# Autodesk Inventor assembly: 42146-00
(part 3 of 3)
- Einfügen:342 [Insert]: 67491-Yellow:12 ↔ 2780-Black:97
- Einfügen:343 [Insert]: 67491-Yellow:12 ↔ 2780-Black:99
- Einfügen:344 [Insert]: 67491-Yellow:12 ↔ 2780-Black:98
- Einfügen:345 [Insert]: 67491-Yellow:12 ↔ 6558-Blue:55
- Einfügen:346 [Insert]: 67491-Yellow:12 ↔ 6558-Blue:56
- Einfügen:347 [Insert]: 67491-Yellow:12 ↔ 6558-Blue:59
- Einfügen:348 [Insert]: 67491-Yellow:12 ↔ 6558-Blue:57
- Einfügen:349 [Insert]: 67491-Yellow:12 ↔ 6558-Blue:58
- Einfügen:350 [Insert]: 42146-20:1 ↔ 67491-Yellow:12
- Passend:154 [Mate]: 42146-20:1 ↔ 6558-Blue:55
- Einfügen:351 [Insert]: 2780-Black:100 ↔ 32525-Yellow:3
- Einfügen:352 [Insert]: 42146-20:1 ↔ 32525-Yellow:4
- Einfügen:353 [Insert]: 42146-20:1 ↔ 32525-Yellow:3
- Einfügen:354 [Insert]: 42146-25:1 ↔ 67491-Yellow:12
- Passend:155 [Mate]: 42146-25:1 ↔ 2780-Black:97
- Einfügen:355 [Insert]: 32054-LtBluishGray:23 ↔ 32524-Yellow:4
- Einfügen:356 [Insert]: 32054-LtBluishGray:24 ↔ 32524-Yellow:6
- Einfügen:357 [Insert]: 2780-Black:101 ↔ 771710-Black:3
- Einfügen:358 [Insert]: 2780-Black:102 ↔ 771710-Black:3
- Einfügen:359 [Insert]: 2780-Black:103 ↔ 771710-Black:3
- Einfügen:360 [Insert]: 6558-Blue:60 ↔ 18654-Black:2
- Einfügen:361 [Insert]: 2780-Black:104 ↔ 32524-Yellow:5
- Einfügen:362 [Insert]: 32524-Yellow:5 ↔ 18654-Black:2
- [Insert]: 6558-Blue:61 ↔ 18654-Black:3
- [Insert]: 2780-Black:105 ↔ 32524-Yellow:7
- [Insert]: 32524-Yellow:7 ↔ 18654-Black:3
- Einfügen:366 [Insert]: 42146-20:1 ↔ 32524-Yellow:4
- Einfügen:367 [Insert]: 42146-20:1 ↔ 32524-Yellow:6
- Passend:156 [Mate]: 42146-25:1 ↔ 32524-Yellow:6
- Passend:157 [Mate]: 42146-25:1 ↔ 32524-Yellow:4
- Einfügen:368 [Insert]: 67491-Yellow:12 ↔ 18654-Black:2
- Einfügen:369 [Insert]: 67491-Yellow:12 ↔ 18654-Black:3
- Einfügen:370 [Insert]: 42146-25:1 ↔ 771710-Black:3
- Passend:158 [Mate]: 42146-25:1 ↔ 2780-Black:101
- Passend:159 [Mate]: 2780-Black:104 ↔ 771710-Black:3
- Passend:160 [Mate]: 771710-Black:3 ↔ 2780-Black:105
- Einfügen:371 [Insert]: 42146-25:1 ↔ 67491-Yellow:13
- Passend:161 [Mate]: 42146-25:1 ↔ 67491-Yellow:13
- Einfügen:372 [Insert]: 771710-Black:1 ↔ 85824 - HUB:1
- Passend:162 [Mate]: 43093-Blue:15 ↔ 85824 - HUB:1
- Passend:163 [Mate]: 42146-24:1 ↔ 84428-LtBluishGray:1
- Passend:164 [Mate] (0.5 mm): 42146-24:1 ↔ 84428-LtBluishGray:1
- Passend:165 [Mate] (0.5 mm): 42146-24:1 ↔ 84428-LtBluishGray:1
- Passend:166 [Mate]: 84428-LtBluishGray:1 ↔ 84428-LtBluishGray:2
- Passend:167 [Mate]: 84428-LtBluishGray:1 ↔ 84428-LtBluishGray:2
- Passend:168 [Mate]: 84428-LtBluishGray:1 ↔ 84428-LtBluishGray:2
- [Mate]: 84428-LtBluishGray:3 ↔ 84428-LtBluishGray:4
- [Mate]: 84428-LtBluishGray:3 ↔ 84428-LtBluishGray:4
- [Mate]: 84428-LtBluishGray:3 ↔ 84428-LtBluishGray:4
- Passend:172 [Mate]: 84428-LtBluishGray:2 ↔ 84428-LtBluishGray:3
- Passend:173 [Mate]: 84428-LtBluishGray:2 ↔ 84428-LtBluishGray:3
- Passend:174 [Mate]: 84428-LtBluishGray:2 ↔ 84428-LtBluishGray:3
- [Mate]: 84428-LtBluishGray:5 ↔ 84428-LtBluishGray:6
- [Mate]: 84428-LtBluishGray:5 ↔ 84428-LtBluishGray:6
- [Mate]: 84428-LtBluishGray:5 ↔ 84428-LtBluishGray:6
- [Mate]: 84428-LtBluishGray:7 ↔ 84428-LtBluishGray:8
- [Mate]: 84428-LtBluishGray:7 ↔ 84428-LtBluishGray:8
- [Mate]: 84428-LtBluishGray:7 ↔ 84428-LtBluishGray:8
- [Mate]: 84428-LtBluishGray:6 ↔ 84428-LtBluishGray:7
- [Mate]: 84428-LtBluishGray:6 ↔ 84428-LtBluishGray:7
- [Mate]: 84428-LtBluishGray:6 ↔ 84428-LtBluishGray:7
- [Mate]: 84428-LtBluishGray:9 ↔ 84428-LtBluishGray:10
- [Mate]: 84428-LtBluishGray:9 ↔ 84428-LtBluishGray:10
- [Mate]: 84428-LtBluishGray:9 ↔ 84428-LtBluishGray:10
- [Mate]: 84428-LtBluishGray:11 ↔ 84428-LtBluishGray:12
- [Mate]: 84428-LtBluishGray:11 ↔ 84428-LtBluishGray:12
- [Mate]: 84428-LtBluishGray:11 ↔ 84428-LtBluishGray:12
- [Mate]: 84428-LtBluishGray:10 ↔ 84428-LtBluishGray:11
- [Mate]: 84428-LtBluishGray:10 ↔ 84428-LtBluishGray:11
- [Mate]: 84428-LtBluishGray:10 ↔ 84428-LtBluishGray:11
- Passend:193 [Mate]: 84428-LtBluishGray:5 ↔ 84428-LtBluishGray:12
- Passend:194 [Mate]: 84428-LtBluishGray:5 ↔ 84428-LtBluishGray:12
- Passend:195 [Mate]: 84428-LtBluishGray:5 ↔ 84428-LtBluishGray:12
- Passend:196 [Mate]: 84428-LtBluishGray:4 ↔ 84428-LtBluishGray:9
- Passend:197 [Mate]: 84428-LtBluishGray:4 ↔ 84428-LtBluishGray:9
- Passend:198 [Mate]: 84428-LtBluishGray:4 ↔ 84428-LtBluishGray:9
- [Mate]: 84428-LtBluishGray:13 ↔ 84428-LtBluishGray:14
- [Mate]: 84428-LtBluishGray:13 ↔ 84428-LtBluishGray:14
- [Mate]: 84428-LtBluishGray:13 ↔ 84428-LtBluishGray:14
- [Mate]: 84428-LtBluishGray:15 ↔ 84428-LtBluishGray:16
- [Mate]: 84428-LtBluishGray:15 ↔ 84428-LtBluishGray:16
- [Mate]: 84428-LtBluishGray:15 ↔ 84428-LtBluishGray:16
- [Mate]: 84428-LtBluishGray:14 ↔ 84428-LtBluishGray:15
- [Mate]: 84428-LtBluishGray:14 ↔ 84428-LtBluishGray:15
- [Mate]: 84428-LtBluishGray:14 ↔ 84428-LtBluishGray:15
- [Mate]: 84428-LtBluishGray:17 ↔ 84428-LtBluishGray:18
- [Mate]: 84428-LtBluishGray:17 ↔ 84428-LtBluishGray:18
- [Mate]: 84428-LtBluishGray:17 ↔ 84428-LtBluishGray:18
- [Mate]: 84428-LtBluishGray:19 ↔ 84428-LtBluishGray:20
- [Mate]: 84428-LtBluishGray:19 ↔ 84428-LtBluishGray:20
- [Mate]: 84428-LtBluishGray:19 ↔ 84428-LtBluishGray:20
- [Mate]: 84428-LtBluishGray:18 ↔ 84428-LtBluishGray:19
- [Mate]: 84428-LtBluishGray:18 ↔ 84428-LtBluishGray:19
- [Mate]: 84428-LtBluishGray:18 ↔ 84428-LtBluishGray:19
- [Mate]: 84428-LtBluishGray:21 ↔ 84428-LtBluishGray:22
- [Mate]: 84428-LtBluishGray:21 ↔ 84428-LtBluishGray:22
- [Mate]: 84428-LtBluishGray:21 ↔ 84428-LtBluishGray:22
- [Mate]: 84428-LtBluishGray:23 ↔ 84428-LtBluishGray:24
- [Mate]: 84428-LtBluishGray:23 ↔ 84428-LtBluishGray:24
- [Mate]: 84428-LtBluishGray:23 ↔ 84428-LtBluishGray:24
- [Mate]: 84428-LtBluishGray:22 ↔ 84428-LtBluishGray:23
- [Mate]: 84428-LtBluishGray:22 ↔ 84428-LtBluishGray:23
- [Mate]: 84428-LtBluishGray:22 ↔ 84428-LtBluishGray:23
- [Mate]: 84428-LtBluishGray:17 ↔ 84428-LtBluishGray:24
- [Mate]: 84428-LtBluishGray:17 ↔ 84428-LtBluishGray:24
- [Mate]: 84428-LtBluishGray:17 ↔ 84428-LtBluishGray:24
- [Mate]: 84428-LtBluishGray:16 ↔ 84428-LtBluishGray:21
- [Mate]: 84428-LtBluishGray:16 ↔ 84428-LtBluishGray:21
- [Mate]: 84428-LtBluishGray:16 ↔ 84428-LtBluishGray:21
- Passend:232 [Mate]: 42146-23:1 ↔ 84428-LtBluishGray:13
- Passend:233 [Mate] (0.5 mm): 42146-23:1 ↔ 84428-LtBluishGray:13
- Passend:234 [Mate] (0.5 mm): 42146-23:1 ↔ 84428-LtBluishGray:13
- Einfügen:373 [Insert]: 6558-Blue:63 ↔ 60484-Yellow:3
- Einfügen:374 [Insert]: 6558-Blue:62 ↔ 60484-Yellow:3
- Einfügen:375 [Insert]: 32073-LtBluishGray:3 ↔ 6536-Yellow:1
- Einfügen:376 [Insert]: 60484-Yellow:3 ↔ 6536-Yellow:1
- Einfügen:377 [Insert]: 60484-Yellow:3 ↔ 6536-Yellow:2
- Passend:235 [Mate]: 32073-LtBluishGray:3 ↔ 6536-Yellow:2
- Einfügen:378 [Insert]: 60484-Yellow:3 ↔ 79768-DkBluishGray:1
- Passend:236 [Mate]: 6558-Blue:63 ↔ 79768-DkBluishGray:1
- [Insert]: 60484-Yellow:4 ↔ 6536-Yellow:3
- Einfügen:380 [Insert]: 79768-DkBluishGray:1 ↔ 60484-Yellow:4
- Passend:237 [Mate]: 6558-Blue:62 ↔ 60484-Yellow:4
- Passend:238 [Mate]: 32073-LtBluishGray:3 ↔ 6536-Yellow:3
- Einfügen:381 [Insert]: 42146-22:1 ↔ 6536-Yellow:1
- Passend:239 [Mate]: 42146-22:1 ↔ 6536-Yellow:3
- Einfügen:382 [Insert]: 42146-22:1 ↔ 77765-MediumStoneGrey:8
- Einfügen:383 [Insert]: 42146-22:1 ↔ 77765-MediumStoneGrey:7
- Einfügen:384 [Insert]: 42146-22:1 ↔ 77765-MediumStoneGrey:9
- Einfügen:385 [Insert]: 42146-22:1 ↔ 32525-LtBluishGray:1
- Passend:240 [Mate]: 42146-22:1 ↔ 32525-LtBluishGray:1
- Einfügen:386 [Insert]: 42146-20:1 ↔ 32054-LtBluishGray:26
- Einfügen:387 [Insert]: 42146-20:1 ↔ 32054-LtBluishGray:25
- Einfügen:388 [Insert]: 42146-20:1 ↔ 42146-26:1
- Einfügen:389 [Insert]: 67498-shock absorber:2 ↔ 2780-Black:106
- Einfügen:390 [Insert]: 67498-shock absorber:2 ↔ 2780-Black:109
- Einfügen:391 [Insert]: 67498-shock absorber:1 ↔ 2780-Black:108
- Einfügen:392 [Insert]: 67498-shock absorber:1 ↔ 2780-Black:107
- Einfügen:393 [Insert]: 67498-shock absorber:2 ↔ 32525-Yellow:3
- Einfügen:394 [Insert]: 67498-shock absorber:1 ↔ 32525-Yellow:4
- Passend:241 [Mate]: 32525-Yellow:4 ↔ 2780-Black:108
- Passend:242 [Mate]: 32525-Yellow:3 ↔ 2780-Black:106
- Passend:243 [Mate]: 42146-26:1 ↔ 67498-shock absorber:2
- Passend:244 [Mate]: 42146-26:1 ↔ 67498-shock absorber:1
- Passend:245 [Mate]: 42146-26:1 ↔ 42146-27:1
- Einfügen:396 [Insert]: 42146-27:1 ↔ 44294-Yellow:1
- Einfügen:397 [Insert]: 42146-27:1 ↔ 44294-Yellow:2
- Einfügen:398 [Insert]: 6632-LtBluishGray:1 ↔ 32062-Red:1
- Einfügen:399 [Insert]: 6632-LtBluishGray:1 ↔ 32062-Red:2
- Einfügen:400 [Insert]: 6632-LtBluishGray:2 ↔ 32062-Red:1
- Passend:246 [Mate]: 6632-LtBluishGray:2 ↔ 32062-Red:2
- Einfügen:401 [Insert]: 2637-LtBluishGray:1 ↔ 6632-LtBluishGray:2
- Fluchtend:4 [Flush]: 2637-LtBluishGray:1 ↔ 6632-LtBluishGray:1
- Fluchtend:5 [Flush]: 2637-LtBluishGray:2 ↔ 6632-LtBluishGray:1
- Einfügen:402 [Insert]: 2637-LtBluishGray:2 ↔ 6632-LtBluishGray:2
- [Insert]: 6632-LtBluishGray:3 ↔ 32062-Red:3
- [Insert]: 6632-LtBluishGray:3 ↔ 32062-Red:4
- [Insert]: 6632-LtBluishGray:4 ↔ 32062-Red:3
- [Mate]: 6632-LtBluishGray:4 ↔ 32062-Red:4
- Einfügen:406 [Insert]: 2637-LtBluishGray:1 ↔ 6632-LtBluishGray:3
- Fluchtend:6 [Flush]: 6632-LtBluishGray:1 ↔ 6632-LtBluishGray:3
- Einfügen:407 [Insert] (-8 mm): 32449-Yellow:1 ↔ 4519-Yellow:1
- Einfügen:408 [Insert]: 32449-Yellow:1 ↔ 32062-Red:5
- Einfügen:409 [Insert]: 32449-Yellow:2 ↔ 32062-Red:5
- Passend:248 [Mate]: 32449-Yellow:2 ↔ 4519-Yellow:1
- Einfügen:410 [Insert]: 2637-LtBluishGray:2 ↔ 32449-Yellow:1
- Fluchtend:7 [Flush]: 6632-LtBluishGray:1 ↔ 32449-Yellow:2
- Einfügen:411 [Insert]: 18942-DkBluishGray:1 ↔ 32449-Yellow:2
- Fluchtend:8 [Flush]: 18942-DkBluishGray:1 ↔ 32449-Yellow:2
- Einfügen:412 [Insert]: 42146-27:1 ↔ 2637-LtBluishGray:3
- Fluchtend:9 [Flush]: 2637-LtBluishGray:1 ↔ 2637-LtBluishGray:3
- Einfügen:413 [Insert] (-36 mm): 3707-Black:1 ↔ 32184-Yellow:1
- Einfügen:414 [Insert] (-36 mm): 32184-Yellow:1 ↔ 3707-Black:2
- Einfügen:415 [Insert]: 2637-LtBluishGray:4 ↔ 32184-Yellow:1
- Einfügen:416 [Insert]: 2637-LtBluishGray:5 ↔ 32184-Yellow:1
- Passend:419 [Mate]: 2637-LtBluishGray:4 ↔ 2637-LtBluishGray:5
- Winkel:4 [Angle] (0 deg): 2637-LtBluishGray:4 ↔ 32184-Yellow:1
- Winkel:5 [Angle] (0 deg): 2637-LtBluishGray:4 ↔ 48989-LtBluishGray:1
- Einfügen:419 [Insert]: 2637-LtBluishGray:5 ↔ 32184-Yellow:2
- Einfügen:420 [Insert]: 2637-LtBluishGray:4 ↔ 32184-Yellow:3
- Passend:251 [Mate]: 3707-Black:2 ↔ 32184-Yellow:3
- Passend:252 [Mate]: 3707-Black:2 ↔ 32184-Yellow:2
- Einfügen:421 [Insert]: 32184-Yellow:3 ↔ 18654-DkBluishGray:2
- Einfügen:422 [Insert]: 32184-Yellow:1 ↔ 18654-DkBluishGray:3
- Einfügen:423 [Insert]: 32184-Yellow:2 ↔ 3713-LtBluishGray:6
- Einfügen:424 [Insert]: 32184-Yellow:3 ↔ 3713-LtBluishGray:5
- Einfügen:425 [Insert]: 32184-Yellow:2 ↔ 32278-LtBluishGray:2
- Einfügen:426 [Insert]: 32184-Yellow:3 ↔ 32278-LtBluishGray:3
- Winkel:6 [Angle] (0 deg): 32184-Yellow:2 ↔ 32278-LtBluishGray:2
- Passend:253 [Mate]: 32278-LtBluishGray:3 ↔ 32278-LtBluishGray:2
- Einfügen:427 [Insert]: 3713-LtBluishGray:6 ↔ 6632-LtBluishGray:5
- Einfügen:428 [Insert]: 3713-LtBluishGray:5 ↔ 6632-LtBluishGray:6
- Passend:254 [Mate]: 3707-Black:2 ↔ 6632-LtBluishGray:6
- Passend:255 [Mate]: 3707-Black:2 ↔ 6632-LtBluishGray:5
- [Insert]: 2637-LtBluishGray:7 ↔ 48989-LtBluishGray:2
- [Insert]: 2637-LtBluishGray:6 ↔ 48989-LtBluishGray:2
- [Angle] (0 deg): 2637-LtBluishGray:6 ↔ 48989-LtBluishGray:2
- Einfügen:431 [Insert]: 48989-LtBluishGray:1 ↔ 2637-LtBluishGray:6
- Passend:256 [Mate]: 48989-LtBluishGray:1 ↔ 2637-LtBluishGray:7
- Winkel:8 [Angle] (0 deg): 48989-LtBluishGray:1 ↔ 48989-LtBluishGray:2
- Einfügen:432 [Insert]: 48989-LtBluishGray:2 ↔ 32524-LtBluishGray:1
- Winkel:9 [Angle] (0 deg): 48989-LtBluishGray:2 ↔ 32524-LtBluishGray:1
- Einfügen:433 [Insert]: 48989-LtBluishGray:2 ↔ 32524-LtBluishGray:2
- Passend:420 [Mate]: 2637-LtBluishGray:4 ↔ 48989-LtBluishGray:1
- Passend:421 [Mate]: 2637-LtBluishGray:4 ↔ 48989-LtBluishGray:1
- Einfügen:435 [Insert]: 79768-DkBluishGray:1 ↔ 6558-Blue:64
- Winkel:10 [Angle] (0 deg): 79768-DkBluishGray:1 ↔ 32524-LtBluishGray:1
- Passend:422 [Mate]: 32524-LtBluishGray:1 ↔ 32524-LtBluishGray:2
- Passend:423 [Mate]: 42146-27:1 ↔ 32278-LtBluishGray:3
- Einfügen:437 [Insert]: 40490-Yellow:1 ↔ 6558-Blue:65
- Einfügen:438 [Insert]: 40490-Yellow:1 ↔ 6558-Blue:66
- [Insert]: 40490-Yellow:2 ↔ 6558-Blue:67
- [Insert]: 40490-Yellow:2 ↔ 6558-Blue:68
- Einfügen:441 [Insert]: 18939-LIGHTGREY:1 ↔ 40490-Yellow:2
- Einfügen:442 [Insert]: 18939-LIGHTGREY:1 ↔ 40490-Yellow:1
- Passend:424 [Mate]: 18939-LIGHTGREY:2 ↔ 6558-Blue:65
- Passend:425 [Mate]: 18939-LIGHTGREY:2 ↔ 6558-Blue:67
- Einfügen:443 [Insert] (0.2 mm): 42146-20:1 ↔ 18939-LIGHTGREY:1
- Einfügen:444 [Insert] (0.2 mm): 42146-20:1 ↔ 18939-LIGHTGREY:2
- Einfügen:445 [Insert]: 42146-28:1 ↔ 18939-LIGHTGREY:1
- Passend:426 [Mate]: 42146-28:1 ↔ 6558-Blue:68
- [Insert]: 6558-Blue:69 ↔ 40490-Yellow:3
- [Insert]: 6558-Blue:70 ↔ 40490-Yellow:3
- [Insert]: 6558-Blue:71 ↔ 40490-Yellow:4
- [Insert]: 6558-Blue:72 ↔ 40490-Yellow:4
- Einfügen:450 [Insert]: 40490-Yellow:3 ↔ 18939-LIGHTGREY:1
- Einfügen:451 [Insert]: 40490-Yellow:4 ↔ 18939-LIGHTGREY:1
- Passend:427 [Mate]: 6558-Blue:70 ↔ 18939-LIGHTGREY:2
- Passend:428 [Mate]: 6558-Blue:72 ↔ 18939-LIGHTGREY:2
- Passend:429 [Mate]: 42146-28:1 ↔ 42146-29:1
- [Insert] (24 mm): 2637-LtBluishGray:8 ↔ 2637-LtBluishGray:9
- [Mate]: 2637-LtBluishGray:8 ↔ 2637-LtBluishGray:9
- [Insert]: 42146-29:1 ↔ 2637-LtBluishGray:8
- [Insert] (-8 mm): 4519-Yellow:3 ↔ 6538c-Red:1
- [Insert] (-8 mm): 4519-Yellow:2 ↔ 6538c-Red:1
- [Insert]: 41677-LtBluishGray:1 ↔ 6538c-Red:1
- [Insert]: 41677-LtBluishGray:2 ↔ 6538c-Red:1
- [Insert] (-8 mm): 4519-Yellow:5 ↔ 6538c-Red:2
- [Insert] (-8 mm): 4519-Yellow:4 ↔ 6538c-Red:2
- [Insert]: 41677-LtBluishGray:2 ↔ 6538c-Red:2
- [Insert]: 43093-Blue:19 ↔ 26287-LtBluishGray:1
- [Insert]: 43093-Blue:20 ↔ 26287-LtBluishGray:1
- [Insert]: 11478-LtBluishGray:1 ↔ 43093-Blue:19
- [Insert]: 32449-Yellow:3 ↔ 11478-LtBluishGray:1
- [Mate]: 32449-Yellow:3 ↔ 11478-LtBluishGray:1
- [Insert]: 41677-LtBluishGray:2 ↔ 11478-LtBluishGray:1
- [Flush]: 41677-LtBluishGray:2 ↔ 32449-Yellow:3
- [Insert] (-8 mm): 11478-LtBluishGray:1 ↔ 32073-LtBluishGray:4
- [Insert]: 32449-Yellow:3 ↔ 32073-LtBluishGray:5
- [Insert]: 11478-LtBluishGray:1 ↔ 42610-LtBluishGray:3
- [Insert]: 42610-LtBluishGray:2 ↔ 42610-LtBluishGray:3
- [Insert]: 42610-LtBluishGray:1 ↔ 42610-LtBluishGray:2
- [Insert]: 41677-LtBluishGray:1 ↔ 2637-LtBluishGray:11
- [Insert]: 41677-LtBluishGray:2 ↔ 2637-LtBluishGray:10
- [Mate]: 2637-LtBluishGray:10 ↔ 2637-LtBluishGray:11
- [Angle] (0 deg): 41677-LtBluishGray:2 ↔ 2637-LtBluishGray:10
- [Insert]: 32449-Yellow:3 ↔ 41677-LtBluishGray:3
- [Flush]: 32449-Yellow:3 ↔ 41677-LtBluishGray:3
- [Insert]: 32449-Yellow:4 ↔ 11478-LtBluishGray:2
- [Mate]: 32449-Yellow:4 ↔ 11478-LtBluishGray:2
- [Insert]: 32449-Yellow:4 ↔ 41677-LtBluishGray:4
- [Flush]: 32449-Yellow:4 ↔ 41677-LtBluishGray:4
- [Insert]: 41677-LtBluishGray:1 ↔ 11478-LtBluishGray:2
- [Mate]: 32073-LtBluishGray:4 ↔ 11478-LtBluishGray:2
- [Insert]: 32062-Red:6 ↔ 92907-LtBluishGray:1
- [Insert]: 32062-Red:7 ↔ 92907-LtBluishGray:1
- [Insert]: 32062-Red:8 ↔ 92907-LtBluishGray:2
- [Insert]: 32062-Red:9 ↔ 92907-LtBluishGray:2
- [Insert]: 2637-LtBluishGray:8 ↔ 92907-LtBluishGray:2
- [Insert]: 2637-LtBluishGray:9 ↔ 92907-LtBluishGray:1
- [Flush]: 92907-LtBluishGray:1 ↔ 92907-LtBluishGray:2
- [Angle] (0 deg): 2637-LtBluishGray:9 ↔ 92907-LtBluishGray:1
- [Insert]: 2637-LtBluishGray:10 ↔ 92907-LtBluishGray:2
- [Angle] (0 deg): 2637-LtBluishGray:11 ↔ 92907-LtBluishGray:1
- Fluchtend:14 [Flush]: 42146-27:1 ↔ 11478-LtBluishGray:1
- Einfügen:485 [Insert]: 42146-29:1 ↔ 44294-Yellow:3
- Einfügen:486 [Insert]: 42146-29:1 ↔ 44294-Yellow:4
- Einfügen:487 [Insert] (-8 mm): 23948-Yellow:1 ↔ 42146-25:1
- Einfügen:488 [Insert] (-72 mm): 80295-White:1 ↔ 23948-Yellow:1
- [Insert]: 42146-29:1 ↔ 64179-Red:2
- [Mate]: 42146-29:1 ↔ 6558-Blue:73
- [Mate]: 42146-31:1 ↔ 42146-32:1
- [Insert]: 4274-Red:1 ↔ 64179-Red:1
- [Insert]: 4274-Red:1 ↔ 58176-TransRed:1
- [Insert]: 42146-30:1 ↔ 64179-Red:1
- [Insert]: 42146-31:1 ↔ 64179-Red:1
- [Insert]: 4274-Red:2 ↔ 58176-TransRed:2
- [Insert]: 64179-Red:2 ↔ 4274-Red:2
- [Insert]: 42146-30:1 ↔ 64179-Red:2
- [Mate]: 42146-31:1 ↔ 64179-Red:2
- [Flush]: 11478-LtBluishGray:4 ↔ 11478-LtBluishGray:6
- [Insert]: 64179-Red:2 ↔ 64179-Red:3
- [Mate]: 64179-Red:1 ↔ 64179-Red:3
- [Insert]: 64179-Red:2 ↔ 6558-Blue:74
- [Insert]: 64179-Red:1 ↔ 6558-Blue:73
- [Insert]: 64179-Red:1 ↔ 11214-Red:13
- [Insert]: 64179-Red:2 ↔ 11214-Red:14
- [Insert]: 64179-Red:2 ↔ 32054-LtBluishGray:30
- [Insert]: 64179-Red:2 ↔ 32054-LtBluishGray:29
- [Insert]: 64179-Red:1 ↔ 32054-LtBluishGray:28
- [Insert]: 64179-Red:1 ↔ 32054-LtBluishGray:27
- [Insert]: 26287-LtBluishGray:2 ↔ 43093-Blue:21
- [Insert]: 26287-LtBluishGray:2 ↔ 43093-Blue:22
- [Insert]: 43093-Blue:21 ↔ 11478-LtBluishGray:3
- [Insert]: 11478-LtBluishGray:3 ↔ 32449-Yellow:5
- [Mate]: 11478-LtBluishGray:3 ↔ 32449-Yellow:5
- [Insert] (-8 mm): 32073-LtBluishGray:6 ↔ 11478-LtBluishGray:3
- [Insert]: 32073-LtBluishGray:7 ↔ 32449-Yellow:5
- [Insert]: 42610-LtBluishGray:6 ↔ 11478-LtBluishGray:3
- [Insert]: 42610-LtBluishGray:6 ↔ 42610-LtBluishGray:5
- [Insert]: 42610-LtBluishGray:5 ↔ 42610-LtBluishGray:4
- [Insert]: 11478-LtBluishGray:4 ↔ 32449-Yellow:6
- [Mate]: 11478-LtBluishGray:4 ↔ 32449-Yellow:6
- [Mate]: 11478-LtBluishGray:4 ↔ 32073-LtBluishGray:6
- [Insert]: 32073-LtBluishGray:8 ↔ 32449-Yellow:6
- [Insert]: 42146-30:1 ↔ 11478-LtBluishGray:4
- [Insert]: 11478-LtBluishGray:4 ↔ 43093-Blue:22
- [Insert]: 43093-Blue:23 ↔ 26287-LtBluishGray:3
- [Insert]: 43093-Blue:24 ↔ 26287-LtBluishGray:3
- [Insert]: 11478-LtBluishGray:5 ↔ 43093-Blue:23
- [Insert]: 32449-Yellow:7 ↔ 11478-LtBluishGray:5
- [Mate]: 32449-Yellow:7 ↔ 11478-LtBluishGray:5
- [Insert] (-8 mm): 11478-LtBluishGray:5 ↔ 32073-LtBluishGray:9
- [Insert]: 32449-Yellow:7 ↔ 32073-LtBluishGray:10
- [Insert]: 11478-LtBluishGray:5 ↔ 42610-LtBluishGray:9
- [Insert]: 42610-LtBluishGray:8 ↔ 42610-LtBluishGray:9
- [Insert]: 42610-LtBluishGray:7 ↔ 42610-LtBluishGray:8
- [Insert]: 32449-Yellow:8 ↔ 11478-LtBluishGray:6
- [Mate]: 32449-Yellow:8 ↔ 11478-LtBluishGray:6
- [Mate]: 32073-LtBluishGray:9 ↔ 11478-LtBluishGray:6
- [Insert]: 43093-Blue:24 ↔ 11478-LtBluishGray:6
- [Insert]: 42146-31:1 ↔ 11478-LtBluishGray:5
- [Insert]: 3706-Red:1 ↔ 41677-LtBluishGray:5
- [Insert]: 32449-Yellow:8 ↔ 41677-LtBluishGray:5
- [Mate]: 32449-Yellow:8 ↔ 3706-Red:1
- [Insert] (-72 mm): 80295-White:2 ↔ 23948-Yellow:2
- Einfügen:536 [Insert]: 80295-White:2 ↔ 42146-20:1
- [Insert]: 3706-Red:2 ↔ 41677-LtBluishGray:6
- Einfügen:538 [Insert]: 41677-LtBluishGray:6 ↔ 3706-Red:1
- Passend:449 [Mate]: 3706-Red:2 ↔ 41677-LtBluishGray:5
- Einfügen:539 [Insert]: 62462-Yellow:1 ↔ 62462-Yellow:2
- Einfügen:540 [Insert]: 3713-LtBluishGray:7 ↔ 62462-Yellow:2
- Einfügen:541 [Insert]: 3713-LtBluishGray:7 ↔ 41677-LtBluishGray:5
- Einfügen:542 [Insert]: 42146-33:1 ↔ 40490-LtBluishGray:2
- Passend:450 [Mate]: 42146-33:1 ↔ 40490-LtBluishGray:2
- Einfügen:543 [Insert]: 42146-34:1 ↔ 40490-LtBluishGray:3
- Passend:451 [Mate]: 42146-34:1 ↔ 40490-LtBluishGray:3
- Einfügen:544 [Insert]: 42146-25:1 ↔ 42146-35:1
- Passend:452 [Mate]: 42146-25:1 ↔ 42146-35:1
- Einfügen:545 [Insert]: 32062-Red:10 ↔ 41677-DKBluishGray:1
- Einfügen:546 [Insert]: 41677-DKBluishGray:1 ↔ 41677-DKBluishGray:2
- Passend:453 [Mate]: 41677-DKBluishGray:1 ↔ 41677-DKBluishGray:2
- Einfügen:547 [Insert]: 41677-DKBluishGray:2 ↔ 25214-LtBluishGray:1
- Winkel:15 [Angle] (0 deg): 41677-DKBluishGray:2 ↔ 25214-LtBluishGray:1
- Einfügen:548 [Insert] (-8 mm): 32054-LtBluishGray:31 ↔ 4519-LtBluishGray:1
- Einfügen:549 [Insert]: 32054-LtBluishGray:31 ↔ 41677-DKBluishGray:1
- Einfügen:550 [Insert]: 41677-DKBluishGray:2 ↔ 25214-LtBluishGray:2
- Winkel:16 [Angle] (0 deg): 41677-DKBluishGray:2 ↔ 25214-LtBluishGray:2
- Einfügen:551 [Insert]: 771710-Black:3 ↔ 32054-LtBluishGray:31
- Winkel:17 [Angle] (0 deg): 771710-Black:3 ↔ 41677-DKBluishGray:2
- Einfügen:552 [Insert]: 42146-36:1 ↔ 67491-Yellow:13
- Passend:454 [Mate]: 42146-36:1 ↔ 67491-Yellow:13
- [Insert]: 4274-Red:6 ↔ 32524-Yellow:8
- [Insert]: 4274-Red:5 ↔ 32524-Yellow:8
- [Insert]: 4274-Red:4 ↔ 32524-Yellow:8
- [Insert]: 4274-Red:3 ↔ 32524-Yellow:8
- Einfügen:557 [Insert]: 42146-34:1 ↔ 32524-Yellow:8
- Passend:455 [Mate]: 42146-34:1 ↔ 32524-Yellow:8
- [Flush]: 4162-LtBluishGray:2 ↔ 4162-LtBluishGray:3
- [Mate]: 4162-LtBluishGray:2 ↔ 4162-LtBluishGray:3
- [Flush]: 4162-LtBluishGray:2 ↔ 4162-LtBluishGray:3
- [Mate]: 4162-LtBluishGray:3 ↔ 3022-Yellow:1
- [Flush]: 4162-LtBluishGray:2 ↔ 3022-Yellow:1
- [Flush]: 4162-LtBluishGray:3 ↔ 3022-Yellow:1
- [Mate]: 4162-LtBluishGray:3 ↔ 3710-Yellow:1
- [Mate]: 3022-Yellow:1 ↔ 3710-Yellow:1
- [Flush]: 3022-Yellow:1 ↔ 3710-Yellow:1
- [Mate]: 4162-LtBluishGray:3 ↔ 2420-Yellow:1
- [Flush]: 3710-Yellow:1 ↔ 2420-Yellow:1
- [Mate]: 3710-Yellow:1 ↔ 2420-Yellow:1
- [Flush]: 4162-LtBluishGray:4 ↔ 4162-LtBluishGray:5
- [Mate]: 4162-LtBluishGray:4 ↔ 4162-LtBluishGray:5
- [Flush]: 4162-LtBluishGray:4 ↔ 4162-LtBluishGray:5
- [Mate]: 3020-Yellow:1 ↔ 3020-Yellow:2
- [Mate]: 3022-Yellow:2 ↔ 3022-Yellow:3
- [Mate]: 4162-LtBluishGray:5 ↔ 3022-Yellow:3
- [Mate]: 4162-LtBluishGray:5 ↔ 3020-Yellow:1
- [Flush]: 4162-LtBluishGray:5 ↔ 3020-Yellow:1
- [Flush]: 4162-LtBluishGray:5 ↔ 3020-Yellow:1
- [Flush]: 3020-Yellow:1 ↔ 3020-Yellow:2
- [Flush]: 3020-Yellow:1 ↔ 3020-Yellow:2
- [Flush]: 4162-LtBluishGray:5 ↔ 3022-Yellow:2
- [Flush]: 3022-Yellow:2 ↔ 3022-Yellow:3
- [Flush]: 3022-Yellow:2 ↔ 3022-Yellow:3
- [Mate] (8 mm): 3022-Yellow:3 ↔ 3020-Yellow:1
- Passend:468 [Mate]: 32524-Yellow:8 ↔ 4162-LtBluishGray:1
- Passend:469 [Mate] (-7.6 mm): 32524-Yellow:8 ↔ 4162-LtBluishGray:1
- Passend:470 [Mate] (-4 mm): 32524-Yellow:8 ↔ 4162-LtBluishGray:1
- Passend:471 [Mate]: 42146-34:1 ↔ 3020-Yellow:2
- Passend:472 [Mate]: 4162-LtBluishGray:1 ↔ 4162-LtBluishGray:4
- Fluchtend:31 [Flush]: 4162-LtBluishGray:1 ↔ 4162-LtBluishGray:4
- Passend:473 [Mate]: 42146-36:1 ↔ 3022-Yellow:1
- Passend:474 [Mate] (-7.6 mm): 42146-36:1 ↔ 3710-Yellow:1
- Fluchtend:32 [Flush]: 42146-36:1 ↔ 2420-Yellow:1
- Einfügen:558 [Insert]: 44873-LtBluishGray:2 ↔ 63037-LtBluishGray:1
- Einfügen:559 [Insert]: 44873-LtBluishGray:1 ↔ 63037-LtBluishGray:2
- Passend:475 [Mate]: 42146-34:1 ↔ 63037-LtBluishGray:2
- Passend:476 [Mate]: 42146-34:1 ↔ 63037-LtBluishGray:1
- Einfügen:560 [Insert] (-5.5 mm): 44873-LtBluishGray:1 ↔ 87994-LtBluishGray:2
- Passend:477 [Mate]: 42146-34:1 ↔ 87994-LtBluishGray:2
- Einfügen:561 [Insert] (-5.5 mm): 44873-LtBluishGray:2 ↔ 87994-LtBluishGray:1
- Passend:478 [Mate]: 87994-LtBluishGray:1 ↔ 44873-LtBluishGray:3
- Einfügen:562 [Insert]: 44873-LtBluishGray:3 ↔ 63965-LtBluishGray:1
- Einfügen:563 [Insert]: 42146-34:1 ↔ 63965-LtBluishGray:1
- Einfügen:564 [Insert]: 4274-LtBluishGray:1 ↔ 32291-DkBluishGray:1
- Einfügen:565 [Insert]: 4274-LtBluishGray:2 ↔ 32291-DkBluishGray:1
- Passend:479 [Mate]: 3023-Black:1 ↔ 32291-DkBluishGray:1
- Passend:480 [Mate]: 4274-LtBluishGray:2 ↔ 3023-Black:1
- Passend:481 [Mate]: 4274-LtBluishGray:1 ↔ 3023-Black:1
- Passend:482 [Mate]: 3023-Black:1 ↔ 54200-TransClear:1
- Passend:483 [Mate]: 3023-Black:1 ↔ 54200-TransClear:2
- Passend:484 [Mate]: 54200-TransClear:1 ↔ 54200-TransClear:2
- Fluchtend:33 [Flush]: 54200-TransClear:1 ↔ 54200-TransClear:2
- Fluchtend:34 [Flush]: 3023-Black:1 ↔ 54200-TransClear:2
- Fluchtend:35 [Flush]: 3023-Black:1 ↔ 54200-TransClear:1
- [Insert]: 4274-LtBluishGray:3 ↔ 32291-DkBluishGray:2
- [Insert]: 4274-LtBluishGray:4 ↔ 32291-DkBluishGray:2
- [Mate]: 3023-Black:2 ↔ 32291-DkBluishGray:2
- [Mate]: 4274-LtBluishGray:4 ↔ 3023-Black:2
- [Mate]: 4274-LtBluishGray:3 ↔ 3023-Black:2
- [Mate]: 3023-Black:2 ↔ 54200-TransClear:3
- [Mate]: 3023-Black:2 ↔ 54200-TransClear:4
- [Mate]: 54200-TransClear:3 ↔ 54200-TransClear:4
- [Flush]: 54200-TransClear:3 ↔ 54200-TransClear:4
- [Flush]: 3023-Black:2 ↔ 54200-TransClear:4
- [Flush]: 3023-Black:2 ↔ 54200-TransClear:3
- Einfügen:568 [Insert]: 43093-Blue:25 ↔ 32291-DkBluishGray:2
- [Insert]: 4274-LtBluishGray:5 ↔ 32291-DkBluishGray:3
- [Insert]: 4274-LtBluishGray:6 ↔ 32291-DkBluishGray:3
- [Mate]: 3023-Black:3 ↔ 32291-DkBluishGray:3
- [Mate]: 4274-LtBluishGray:6 ↔ 3023-Black:3
- [Mate]: 4274-LtBluishGray:5 ↔ 3023-Black:3
- [Mate]: 3023-Black:3 ↔ 54200-TransClear:5
- [Mate]: 3023-Black:3 ↔ 54200-TransClear:6
- [Mate]: 54200-TransClear:5 ↔ 54200-TransClear:6
- [Flush]: 54200-TransClear:5 ↔ 54200-TransClear:6
- [Flush]: 3023-Black:3 ↔ 54200-TransClear:6
- [Flush]: 3023-Black:3 ↔ 54200-TransClear:5
- [Insert]: 43093-Blue:26 ↔ 32291-DkBluishGray:3
- Einfügen:572 [Insert]: 32291-DkBluishGray:1 ↔ 43093-Blue:27
- Einfügen:573 [Insert]: 42146-34:1 ↔ 43093-Blue:26
- Winkel:18 [Angle] (0 deg): 42146-34:1 ↔ 3023-Black:3
- Einfügen:574 [Insert]: 42146-28:1 ↔ 43093-Blue:27
- Einfügen:575 [Insert]: 42146-28:1 ↔ 43093-Blue:25
- Fluchtend:42 [Flush]: 3023-Black:1 ↔ 3023-Black:2
- Passend:497 [Mate]: 42146-28:1 ↔ 32291-DkBluishGray:2
- Einfügen:576 [Insert] (-72 mm): 80295-White:4 ↔ 23948-Yellow:3
- Einfügen:577 [Insert] (8 mm): 80295-White:3 ↔ 80295-White:4
- Einfügen:578 [Insert] (-8 mm): 23948-Yellow:3 ↔ 42146-25:1
- Passend:498 [Mate] (-4 mm): 42146-30:1 ↔ 42146-37:1
- Passend:499 [Mate] (-400 mm): 42146-37:1 ↔ 40490-LtBluishGray:1
- Passend:500 [Mate] (10.838 mm): 42146-30:1 ↔ 42146-37:1
- Passend:501 [Mate] (12 mm): 42146-38:1 ↔ 42146-20:1
- Passend:502 [Mate]: 42146-38:1 ↔ 23948-Yellow:1
- Winkel:20 [Angle] (0 deg): 42146-38:1 ↔ 42146-20:1
- Passend:503 [Mate] (8 mm): 42146-39:1 ↔ 42146-20:1
- Passend:504 [Mate]: 42146-39:1 ↔ 23948-Yellow:2
- Winkel:21 [Angle] (0 deg): 42146-39:1 ↔ 42146-20:1
- Passend:505 [Mate] (-4 mm): 42146-40:1 ↔ 42146-20:1
- Passend:506 [Mate]: 42146-40:1 ↔ 23948-Yellow:3
- Winkel:22 [Angle] (0 deg): 42146-40:1 ↔ 42146-20:1
- [Insert] (-12 mm): 32062-Red:11 ↔ 6536-Yellow:4
- [Insert] (-12 mm): 32062-Red:12 ↔ 6536-Yellow:5
- [Insert]: 6536-Yellow:4 ↔ 6632-LtBluishGray:8
- [Insert]: 6536-Yellow:4 ↔ 6632-LtBluishGray:7
- [Insert]: 6632-LtBluishGray:8 ↔ 6536-Yellow:5
- [Mate]: 6632-LtBluishGray:8 ↔ 32062-Red:12
- [Mate]: 32062-Red:11 ↔ 6632-LtBluishGray:8
- [Mate]: 6632-LtBluishGray:7 ↔ 32062-Red:12
- [Insert]: 42146-30:1 ↔ 6632-LtBluishGray:7
- [Insert]: 42146-30:1 ↔ 77765-MediumStoneGrey:10
- [Insert]: 42610-LtBluishGray:10 ↔ 6536-Yellow:5
- [Insert]: 6536-Yellow:4 ↔ 77765-MediumStoneGrey:11
- Winkel:23 [Angle] (0 deg): 42146-37:1 ↔ 6632-LtBluishGray:8
## Named parameters: d58_d57 = 7.2 mm, d67_d66 = 0 mm, d68_d65 = 0 mm, d101_d97 = 0 mm, d102_d98 = 0 mm, d103_d99 = 0 mm, d104_d100 = 0 mm, d121_d114 = 0 mm, d122_d115 = 0 mm, d123_d116 = 0 mm, d164_d153 = 0 mm, d165_d154 = 0 mm, d166_d155 = 0 mm, d167_d156 = 0 mm, d168_d157 = 0 mm, d209_d154 = 0 mm, d210_d155 = 0 mm, d211_d156 = 0 mm, d212_d157 = 0 mm, d217_d198 = 0 mm, d218_d199 = 0 mm, d219_d200 = 0 mm, d220_d201 = 0 mm, d221_d202 = 0 mm, d222_d203 = 0 mm, d223_d204 = 0 mm, d224_d205 = 0 mm, d225_d209_d154 = 0 mm, d226_d210_d155 = 0 mm, d227_d211_d156 = 0 mm, d228_d212_d157 = 0 mm, d229_d213 = 0 mm, d230_d214 = 0 mm, d231_d179 = 0 mm, d232_d180 = 0 mm, d233_d181 = 0 mm, d234_d182 = 0 mm, d235_d183 = 0 mm, d236_d186 = 0 mm, d237_d187 = 0 mm, d238_d188 = 0 mm, d239_d189 = 0 mm, d240_d190 = 0 mm, d241_d191 = 0 mm, d242_d192 = 0 mm, d243_d193 = 0 mm, d244_d194 = 0 mm, d245_d195 = 0 mm, d246_d196 = 0 mm, d247_d197 = 7.2 mm, d248_d175 = 0 mm, d249_d176 = 0 mm, d250_d177 = 7.2 mm, d251_d178 = 0 mm, d264_d209_d154 = 0 mm, d265_d210_d155 = 0 mm, d266_d211_d156 = 0 mm, d267_d212_d157 = 0 mm, d270_d225_d209_d154 = 0 mm, d271_d226_d210_d155 = 0 mm, d272_d227_d211_d156 = 0 mm, d273_d228_d212_d157 = 0 mm, d357_d354 = 0 mm, d358_d355 = 0 mm, d359_d356 = 0 mm, d364_d318 = 0 mm, d365_d319 = 0 mm, d368_d364_d318 = 0 mm, d369_d365_d319 = 0 mm, d370_d366 = 0 mm, d371_d367 = 0 mm, d393_d390 = 0 mm, d394_d391 = 0 mm, d395_d392 = 0 mm, d404_d402 = 0 mm, d405_d403 = 0 mm, d435_d433 = 0 mm, d436_d434 = 0 mm, d449_d446 = 0 mm, d465_d379 = 0 mm, d481_d479 = 0 mm, d482_d480 = 0 mm, d483_d479 = 0 mm, d484_d480 = 0 mm, d485_d479 = 0 mm, d486_d480 = 0 mm, d495_d465_d379 = 0 mm, d517_d516 = 0 mm, d524_d521 = 0 mm, d525_d522 = 0 mm, d526_d523 = 0 mm, d547_d544 = 0 mm, d548_d545 = 0 mm, d549_d546 = 0 mm, d553_d544 = 0 mm, d554_d545 = 0 mm, d555_d546 = 0 mm, d556_d547_d544 = 0 mm, d557_d548_d545 = 0 mm, d558_d549_d546 = 0 mm, d559_d550 = 0 mm, d560_d551 = 0 mm, d561_d552 = 0 mm, d562_d544 = 0 mm, d563_d545 = 0 mm, d564_d546 = 0 mm, d565_d547_d544 = 0 mm, d566_d548_d545 = 0 mm, d567_d549_d546 = 0 mm, d568_d550 = 0 mm, d569_d551 = 0 mm, d570_d552 = 0 mm, d577_d544 = 0 mm, d578_d545 = 0 mm, d579_d576 = 0 mm, d580_d546 = 0 mm, d581_d547_d544 = 0 mm, d582_d548_d545 = 0 mm, d583_d549_d546 = 0 mm, d584_d550 = 0 mm, d585_d551 = 0 mm, d586_d552 = 0 mm, d587_d553_d544 = 0 mm, d588_d554_d545 = 0 mm, d589_d555_d546 = 0 mm, d590_d556_d547_d544 = 0 mm, d591_d557_d548_d545 = 0 mm, d592_d558_d549_d546 = 0 mm, d593_d559_d550 = 0 mm, d594_d560_d551 = 0 mm, d595_d561_d552 = 0 mm, d596_d562_d544 = 0 mm, d597_d563_d545 = 0 mm, d598_d564_d546 = 0 mm, d599_d565_d547_d544 = 0 mm, d600_d566_d548_d545 = 0 mm, d601_d567_d549_d546 = 0 mm, d602_d568_d550 = 0 mm, d603_d569_d551 = 0 mm, d604_d570_d552 = 0 mm, d605_d571 = 0 mm, d606_d572 = 0 mm, d607_d573 = 0 mm, d608_d574 = 0 mm, d609_d575 = 0 mm, d621_d616 = 0 mm, d657_d649 = 0 mm, d658_d650 = 0 mm, d659_d651 = 0 mm, d660_d652 = 0 mm, d699_d679 = 0 mm, d700_d680 = 0 mm, d701_d682 = 0 deg, d718_d716 = 0 mm, d719_d717 = 0 mm, d728_d718_d716 = 0 mm, d729_d719_d717 = 0 mm, d730_d718_d716 = 0 mm, d731_d719_d717 = 0 mm, d738_d134 = 0 mm, d739_d135 = 0 deg, d740_d136 = 0 mm, d741_d137 = 0 deg, d742_d112 = 0 mm, d743_d113 = 0 mm, d744_d114 = 0 mm, d745_d115 = 0 mm, d746_d116 = 0 mm, d747_d117 = 0 mm, d748_d118 = 0 mm, d749_d119 = 0 deg, d750_d120 = 0 mm, d122_d107 = 0 mm, d123_d108 = 0 mm, d124_d121 = 0 mm, d125_d120 = 0 mm, d756_d126 = 0 mm, d757_d127 = 0 mm, d758_d128 = 0 mm, d759_d129 = 0 mm, d130_d128 = 0 mm, d131_d129 = 0 mm, d762_d132 = 0 mm, d763_d133 = 0 mm, d764_d97 = -8 mm, d765_d98 = -8 mm, d766_d99 = 0 mm, d767_d100 = 0 mm, d768_d101_d97 = -8 mm, d769_d102_d98 = -8 mm, d772_d105 = 0 mm, d773_d106 = 0 mm, d774_d107 = 0 mm, d775_d108 = 0 mm, d776_d109 = 0 mm, d777_d110 = 0 mm, d778_d111 = -8 mm, d779_d90 = 24 mm, d780_d91 = 0 mm, d781_d92 = 0 mm, d792_d5 = 0 mm, d6_d3 = 0 mm, d794_d7 = 0 mm, d795_d8 = 0 mm, d796_d9 = 0 mm, d798_d11 = 0 mm, d799_d12 = 0 mm, d800_d13 = 0 mm, d801_d14 = 0 mm, d802_d15 = 0 mm, d803_d16 = 0 mm, d804_d17 = 0 mm, d805_d18 = 0 mm, d806_d19 = 0 mm, d807_d20 = 0 mm, d808_d21 = 0 mm, d810_d2 = 0 mm, d811_d3 = 0 mm, d812_d4 = 0 mm, d814_d742_d112 = 0 mm, d815_d743_d113 = 0 mm, d816_d744_d114 = 0 mm, d817_d745_d115 = 0 mm, d818_d122_d107 = 0 mm, d819_d123_d108 = 0 mm, d820_d757_d127 = 0 mm, d821_d104 = 0 mm, d822_d772_d105 = 0 mm, d823_d773_d106 = 0 mm, d824_d774_d107 = 0 mm, d825_d775_d108 = 0 mm, d826_d778_d111 = -8 mm, d827_d20 = 0 mm, d828_d23 = 0 mm, d829_d24 = 0 mm, d830_d31 = 0 mm, d831_d32 = 0 mm, d832_d33 = 0 mm, d833_d742_d112 = 0 mm, d834_d743_d113 = 0 mm, d835_d744_d114 = 0 mm, d836_d745_d115 = 0 mm, d837_d122_d107 = 0 mm, d838_d123_d108 = 0 mm, d839_d757_d127 = 0 mm, d840_d104 = 0 mm, d841_d772_d105 = 0 mm, d842_d773_d106 = 0 mm, d843_d774_d107 = 0 mm, d844_d775_d108 = 0 mm, d845_d778_d111 = -8 mm, d846_d24 = 0 mm, d847_d21 = 0 mm, d849_d787 = -72 mm, d851_d830_d31 = 0 mm, d877_d24 = 0 mm, d878_d25 = 0 mm, d879_d21 = 0 mm, d880_d22 = 0 mm, d883_d1 = 0 mm, d884_d2 = 0 mm, d885_d3 = 0 mm, d886_d4 = 0 mm, d887_d5 = 0 mm, d888_d6 = 0 mm, d889_d7 = 0 mm, d890_d8 = 0 mm, d891_d9 = 0 mm, d892_d10 = 0 mm, d893_d11 = 0 mm, d12_d1 = 0 mm, d13_d2 = 0 mm, d14_d0 = 0 mm, d897_d0 = 0 mm, d898_d15 = 0 mm, d899_d16 = 0 mm, d900_d17 = 0 mm, d901_d18 = 0 mm, d902_d19 = 0 mm, d903_d20 = 0 mm, d904_d21 = 0 mm, d905_d22 = 0 mm, d906_d23 = 0 mm, d907_d24 = 0 mm, d908_d25 = 0 mm, d909_d26 = 8 mm, d940_d929 = 0 mm, d941_d930 = 0 mm, d942_d931 = 0 mm, d943_d932 = 0 mm, d944_d933 = 0 mm, d945_d934 = 0 mm, d946_d935 = 0 mm, d947_d936 = 0 mm, d948_d937 = 0 mm, d949_d938 = 0 mm, d950_d939 = 0 mm, d952_d940_d929 = 0 mm, d953_d941_d930 = 0 mm, d954_d942_d931 = 0 mm, d955_d943_d932 = 0 mm, d956_d944_d933 = 0 mm, d957_d945_d934 = 0 mm, d958_d946_d935 = 0 mm, d959_d947_d936 = 0 mm, d960_d948_d937 = 0 mm, d961_d949_d938 = 0 mm, d962_d950_d939 = 0 mm, d963_d951 = 0 mm, d990_d162 = 0 mm, d991_d151 = -12 mm, d152_d151 = -12 mm, d993_d153 = 0 mm, d994_d154 = 0 mm, d995_d155 = 0 mm, d996_d156 = 0 mm, d997_d157 = 0 mm, d998_d158 = 0 mm, d999_d159 = 0 mm
